# Autodesk Inventor assembly: final
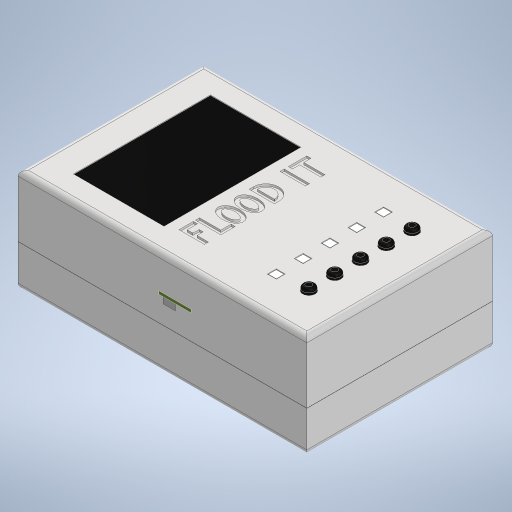
[picture p0: Inventor's stored thumbnail of the model, 512x512]
Saved by Autodesk Inventor 2023 (Build 270158000, 158)
## iProperties
Created: 2022-12-09
Part Number: final
Document SubType Name: Assembly
Designer: spfow
Author: spfow
## Documents named in this file (10)
- C:\Users\spfow\OneDrive\Documents\ECE_414\Final_Project\CAD\final.iam
- C:\Users\spfow\OneDrive\Documents\ECE_414\Final_Project\CAD\Audio_jack.ipt
- C:\Users\spfow\OneDrive\Documents\ECE_414\Final_Project\CAD\CaseBottom.ipt
- C:\Users\spfow\OneDrive\Documents\ECE_414\Final_Project\CAD\CaseTop2.0.ipt
- C:\Users\spfow\OneDrive\Documents\ECE_414\Final_Project\CAD\LCD_Display.ipt
- C:\Users\spfow\OneDrive\Documents\ECE_414\Final_Project\CAD\LED_Strip.ipt
- C:\Users\spfow\OneDrive\Documents\ECE_414\Final_Project\CAD\Button_switch.ipt
- C:\Users\spfow\OneDrive\Documents\ECE_414\Final_Project\CAD\micro1.ipt
- C:\Users\spfow\OneDrive\Documents\ECE_414\Final_Project\CAD\micro2.ipt
- C:\Users\spfow\OneDrive\Documents\ECE_414\Final_Project\CAD\Battery Cover2.0.ipt
## Components (13 placed, 9 different names)
1. Audio_jack:1 — Mate:3, Mate:4, Mate:5
2. CaseBottom:1 — Insert:6, Insert:7, Flush:5, Mate:14
3. CaseTop2.0:1 — Mate:3, Mate:4, Mate:5, Insert:1, Insert:2, Insert:3, Insert:4, Insert:5, Flush:1, Mate:6, Mate:7, Flush:2, Mate:8, Mate:9, Insert:6, Insert:7, Mate:10, Mate:11, Flush:3, Flush:4, Mate:12, Mate:13
4. Button_switch:1 — Insert:5
5. Button_switch:2 — Insert:1
6. Button_switch:3 — Insert:3
7. Button_switch:4 — Insert:2
8. Button_switch:5 — Insert:4
9. LED_Strip:1 — Flush:1, Mate:6, Mate:7
10. LCD_Display:1 — Flush:2, Mate:8, Mate:9
11. micro1:1 — Mate:10, Mate:11, Flush:3
12. micro2:1 — Flush:4, Mate:12, Mate:13
13. Battery Cover2.0:1 — Flush:5, Mate:14
## Relationships (24: Mate 12, Insert 7, Flush 5)
- Mate:3: Audio_jack:1 ↔ CaseTop2.0:1
- Mate:4: Audio_jack:1 ↔ CaseTop2.0:1
- Mate:5: Audio_jack:1 ↔ CaseTop2.0:1
- Insert:1: CaseTop2.0:1 ↔ Button_switch:2
- Insert:2: CaseTop2.0:1 ↔ Button_switch:4
- Insert:3: CaseTop2.0:1 ↔ Button_switch:3
- Insert:4: CaseTop2.0:1 ↔ Button_switch:5
- Insert:5: CaseTop2.0:1 ↔ Button_switch:1
- Flush:1: CaseTop2.0:1 ↔ LED_Strip:1
- Mate:6 (0.254 mm): CaseTop2.0:1 ↔ LED_Strip:1
- Mate:7 (0.254 mm): CaseTop2.0:1 ↔ LED_Strip:1
- Flush:2: CaseTop2.0:1 ↔ LCD_Display:1
- Mate:8: CaseTop2.0:1 ↔ LCD_Display:1
- Mate:9: CaseTop2.0:1 ↔ LCD_Display:1
- Insert:6: CaseBottom:1 ↔ CaseTop2.0:1
- Insert:7: CaseBottom:1 ↔ CaseTop2.0:1
- Mate:10: CaseTop2.0:1 ↔ micro1:1
- Mate:11: CaseTop2.0:1 ↔ micro1:1
- Flush:3: CaseTop2.0:1 ↔ micro1:1
- Flush:4: CaseTop2.0:1 ↔ micro2:1
- Mate:12: CaseTop2.0:1 ↔ micro2:1
- Mate:13: CaseTop2.0:1 ↔ micro2:1
- Flush:5: CaseBottom:1 ↔ Battery Cover2.0:1
- Mate:14: CaseBottom:1 ↔ Battery Cover2.0:1
